# Autodesk Inventor assembly: KelleWelle.ipt
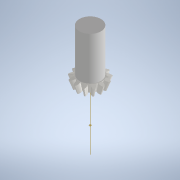
[picture p0: Inventor's stored thumbnail of the model, 180x180]
Saved by Autodesk Inventor 2021 (Build 250183000, 183)
## iProperties
Created: 2021-01-29
Part Number: KelleWelle.ipt
Document SubType Name: Assembly
Designer: LETPJG
Author: LETPJG
## Documents named in this file (3)
- C:\Users\LETPJG\Documents\Vault\Gruppen\Gruppe 2\Entwurf\Amphibienfahrzeug\KelleWelle.ipt.iam
- C:\Users\LETPJG\Documents\Vault\Gruppen\Gruppe 2\Entwurf\Amphibienfahrzeug\Kegelräder16_MIR.iam
- C:\Users\LETPJG\Documents\Vault\Gruppen\Gruppe 2\Entwurf\Amphibienfahrzeug\BauteilWelle1.ipt
## Components (2 placed, 2 different names)
1. Kegelräder16_MIR:1 [sub-assembly] — Einfügen:1
2. BauteilWelle1:1 — Einfügen:1
## Relationships (1: Insert 1)
- Einfügen:1 [Insert]: Kegelräder16_MIR:1 ↔ BauteilWelle1:1
